# Autodesk Inventor assembly: translationStageAssembly
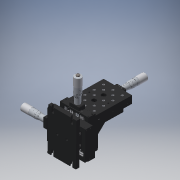
[picture p0: Inventor's stored thumbnail of the model, 180x180]
Saved by Autodesk Inventor 2016 (Build 200138000, 138)
## iProperties
Created: 2016-03-16
Part Number: translationStageAssembly
Document SubType Name: Assembly
Designer: sims01
Author: sims01
## Documents named in this file (4)
- H:\Documents\LSFM_3\setup\mechanical\design\lsfm3_mechDesignMar16\translationStageAssembly.iam
- H:\Documents\LSFM_3\setup\mechanical\design\purchasedComponents\translationStagePt1.ipt
- H:\Documents\LSFM_3\setup\mechanical\design\purchasedComponents\translationStagePt2.ipt
- H:\Documents\LSFM_3\setup\mechanical\design\purchasedComponents\translationStagePt3.ipt
## Components (5 placed, 3 different names)
1. translationStagePt1:1 — Rigid:1, Rigid:2
2. translationStagePt1:2 — Rigid:3
3. translationStagePt1:3 — Rigid:1
4. translationStagePt2:1
5. translationStagePt3:1 — Rigid:2, Rigid:3
## Relationships (3: WeldJoint 3)
- Rigid:1 [WeldJoint]: translationStagePt1:1 ↔ translationStagePt1:3
- Rigid:2 [WeldJoint]: translationStagePt1:1 ↔ translationStagePt3:1
- Rigid:3 [WeldJoint]: translationStagePt1:2 ↔ translationStagePt3:1
